# Autodesk Inventor assembly: Ensamblaje2
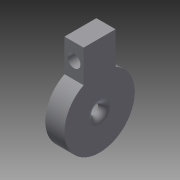
[picture p0: Inventor's stored thumbnail of the model, 180x180]
Saved by Autodesk Inventor 2015 SP1 (Build 190203100, 203)
## iProperties
Created: 2015-07-03
Part Number: Ensamblaje2
Document SubType Name: Assembly
Designer: Javier
Author: Javier
## Documents named in this file (4)
- D:\Dropbox\3dprint\riego\Ensamblaje2.iam
- D:\Dropbox\3dprint\riego\valvula-cocacola-v1.ipt
- D:\Dropbox\3dprint\riego\soporte-servo-valvula.ipt
- D:\Dropbox\3dprint\riego\enganche-servo-cable.ipt
## Components (3 placed, 3 different names)
1. valvula-cocacola-v1:1 — Nivelación:1
2. soporte-servo-valvula:1 — Nivelación:1
3. enganche-servo-cable:1
## Relationships (1: Flush 1)
- Nivelación:1 [Flush]: valvula-cocacola-v1:1 ↔ soporte-servo-valvula:1
